# Autodesk Inventor assembly: ABD_MX_64_Slider_Fixation_Set_Right2Horn
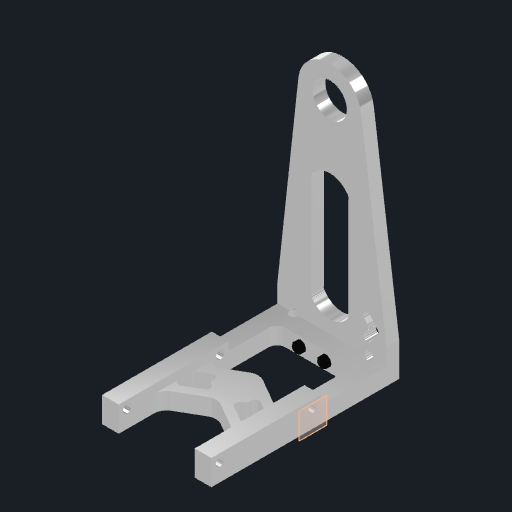
[picture p0: Inventor's stored thumbnail of the model, 512x512]
Saved by Autodesk Inventor 2024 (Build 280153000, 153)
## iProperties
Created: 2024-02-15
Part Number: ABD_MX_64_Slider_Fixation_Set_Right2Horn
Document SubType Name: Assembly
Designer: ASUS
Author: ASUS
## Documents named in this file (4)
- C:\Users\ASUS\Desktop\Anti_Backlash_Structure_OP\v2_Frame\ABD_MX_64_Slider_Fixation_Set_Right2Horn.iam
- C:\Users\ASUS\Desktop\Anti_Backlash_Structure_OP\v2_Frame\106_Slider_Fixation_MIR.ipt
- C:\Users\ASUS\Desktop\Anti_Backlash_Structure_OP\MISUMI\CSH-ST-M2_5-8_203.ipt
- C:\Users\ASUS\Desktop\Anti_Backlash_Structure_OP\v2_Frame\Leg_joint_slider_frame_v2.ipt
## Components (4 placed, 3 different names)
1. 106_Slider_Fixation_MIR:1 — 삽입:3, 메이트:1
2. CSH-ST-M2_5-8_203:2 — 삽입:1
3. Leg_joint_slider_frame_v2:1 — 삽입:1, 삽입:3, 삽입:4
4. CSH-ST-M2_5-8_203:3 — 삽입:4, 메이트:1
## Relationships (4: Insert 3, Mate 1)
- 삽입:1 [Insert]: CSH-ST-M2_5-8_203:2 ↔ Leg_joint_slider_frame_v2:1
- 삽입:3 [Insert]: 106_Slider_Fixation_MIR:1 ↔ Leg_joint_slider_frame_v2:1
- 삽입:4 [Insert]: Leg_joint_slider_frame_v2:1 ↔ CSH-ST-M2_5-8_203:3
- 메이트:1 [Mate]: 106_Slider_Fixation_MIR:1 ↔ CSH-ST-M2_5-8_203:3
